# Autodesk Inventor assembly: Grundplatte_test
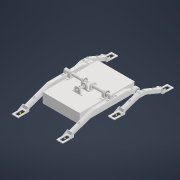
[picture p0: Inventor's stored thumbnail of the model, 180x180]
Saved by Autodesk Inventor 2021 (Build 250183000, 183)
## iProperties
Created: 2021-01-26
Part Number: Grundplatte_test
Document SubType Name: Assembly
Designer: Ctroi
Author: Ctroi
## Documents named in this file (22)
- G:\Roverprojekt\Github Projekt\Rover\Grundplatte_test.iam
- G:\Roverprojekt\Github Projekt\Rover\Grundplatte_hinten.ipt
- G:\Roverprojekt\Github Projekt\Rover\Grundplatte_vorne.ipt
- G:\Roverprojekt\Github Projekt\Rover\ArduinoMega.ipt
- G:\Roverprojekt\Github Projekt\Rover\Relais.ipt
- G:\Roverprojekt\Github Projekt\Rover\Kreuz_Halterung.ipt
- G:\Roverprojekt\Github Projekt\Rover\Obenplatte_hinten.ipt
- G:\Roverprojekt\Github Projekt\Rover\Obenplatte_vorne.ipt
- G:\Roverprojekt\Github Projekt\Rover\Halterung_Differential_3.ipt
- G:\Roverprojekt\Github Projekt\Rover\Halterung_Differential_Mitte.ipt
- G:\Roverprojekt\Github Projekt\Rover\Halterung_Differential.ipt
- G:\Roverprojekt\Github Projekt\Rover\Halterung_Differential_2.ipt
- G:\Roverprojekt\Github Projekt\Rover\Kugellager.ipt
- G:\Roverprojekt\Github Projekt\Rover\Kugellager_klein.ipt
- G:\Roverprojekt\Github Projekt\Rover\Verbindung_Rocker_Body.ipt
- G:\Roverprojekt\Github Projekt\Rover\Welle_Kugellager_Mitte.ipt
- G:\Roverprojekt\Github Projekt\Rover\Rocker_hinten_rechts.ipt
- G:\Roverprojekt\Github Projekt\Rover\Rocker_hinten.ipt
- G:\Roverprojekt\Github Projekt\Rover\Rocker_vorne.ipt
- G:\Roverprojekt\Github Projekt\Rover\Bogie.ipt
- G:\Roverprojekt\Github Projekt\Rover\Boogie_Stange.ipt
- G:\Roverprojekt\Github Projekt\Rover\Servohalterung_v2.ipt
## Components (40 placed, 20 different names)
1. Fahrwerk_bogie:1 — Passend:70, Passend:71, Fluchtend:5, Fluchtend:6, Passend:72, Fluchtend:7, Fluchtend:8, Passend:73
2. Fahrwerk_bogie:2 — Passend:68, Passend:69, Fluchtend:13, Fluchtend:14, Passend:76, Fluchtend:15, Fluchtend:16, Passend:77
3. Boogie_Stange:1 — Passend:64, Passend:65, Passend:68, Passend:69
4. Boogie_Stange:2 — Passend:66, Passend:67, Passend:70, Passend:71
5. Servohalterung_v2:1 — Fluchtend:9, Fluchtend:10, Passend:74
6. Servohalterung_v2:2 — Fluchtend:11, Fluchtend:12, Passend:75
7. Servohalterung_v2:3 — Fluchtend:13, Fluchtend:14, Passend:76
8. Servohalterung_v2:4 — Fluchtend:7, Fluchtend:8, Passend:73
9. Servohalterung_v2:5 — Fluchtend:15, Fluchtend:16, Passend:77
10. Servohalterung_v2:6 — Fluchtend:5, Fluchtend:6, Passend:72
11. Grundplatte_hinten:1 — Passend:1, Passend:2, Passend:5, Passend:6, Passend:7, Passend:11, Passend:12, Passend:13, Passend:16
12. Grundplatte_vorne:1 — Passend:1, Passend:2, Passend:3, Passend:4, Passend:8, Passend:9, Passend:10, Passend:16
13. ArduinoMega:1 — Passend:3, Passend:4
14. Relais:1
15. Kreuz_Halterung:1 — Passend:5, Passend:6, Passend:7
16. Welle_Kugellager_Mitte:1 — Passend:48, Passend:49
17. Obenplatte_vorne:1 — Passend:8, Passend:9, Passend:10, Passend:15, Passend:17, Passend:18, Passend:21, Passend:22, Passend:23, Passend:24, Passend:27, Passend:28
18. Halterung_Differential_3:1 — Passend:14, Passend:15, Passend:17, Passend:38, Passend:39
19. Halterung_Differential_3:2 — Passend:18, Passend:19, Passend:20, Passend:32, Passend:33
20. Obenplatte_hinten:1 — Passend:11, Passend:12, Passend:13, Passend:14, Passend:19, Passend:20, Passend:25, Passend:26
21. Halterung_Differential_Mitte:1 — Passend:21, Passend:22, Passend:23, Passend:42, Passend:43
22. Halterung_Differential:1 — Passend:26, Passend:27, Passend:28, Passend:30, Passend:31, Passend:36, Passend:37
23. Halterung_Differential:2 — Passend:24, Passend:25, Passend:29, Passend:34, Passend:35
24. Halterung_Differential_2:1 — Passend:29, Passend:30, Passend:31, Passend:40, Passend:41
25. Kugellager:1 — Passend:40, Passend:41, Passend:48, Passend:49
26. Kugellager:2 — Passend:32, Passend:33, Passend:47
27. Kugellager:3 — Passend:34, Passend:35, Passend:44
28. Kugellager:4 — Passend:36, Passend:37, Passend:45
29. Kugellager:5 — Passend:38, Passend:39, Passend:46
30. Kugellager_klein:1 — Passend:42, Passend:43
31. Fahrwerk_rocker_vorne:1 — Fluchtend:1, Fluchtend:2, Passend:62, Fluchtend:11, Fluchtend:12, Passend:75
32. Kugellager:7 — Passend:54, Passend:55, Passend:64, Passend:65
33. Kugellager:6 — Passend:52, Passend:53
34. Fahrwerk_rocker_hinten:1 — Passend:50, Passend:51, Passend:52, Passend:53, Passend:54, Passend:55, Fluchtend:1, Fluchtend:2, Passend:62
35. Verbindung_Rocker_Body:1 — Passend:44, Passend:47, Passend:50, Passend:51
36. Kugellager:9 — Passend:60, Passend:61
37. Kugellager:8 — Passend:58, Passend:59, Passend:66, Passend:67
38. Fahrwerk_rocker_hinten:2 — Passend:56, Passend:57, Passend:58, Passend:59, Passend:60, Passend:61, Fluchtend:3, Fluchtend:4, Passend:63
39. Fahrwerk_rocker_vorne:2 — Fluchtend:3, Fluchtend:4, Passend:63, Fluchtend:9, Fluchtend:10, Passend:74
40. Verbindung_Rocker_Body:2 — Passend:45, Passend:46, Passend:56, Passend:57
## Relationships (93: Mate 77, Flush 16)
- Passend:1 [Mate]: Grundplatte_hinten:1 ↔ Grundplatte_vorne:1
- Passend:2 [Mate]: Grundplatte_hinten:1 ↔ Grundplatte_vorne:1
- Passend:3 [Mate]: Grundplatte_vorne:1 ↔ ArduinoMega:1
- Passend:4 [Mate]: Grundplatte_vorne:1 ↔ ArduinoMega:1
- Passend:5 [Mate]: Grundplatte_hinten:1 ↔ Kreuz_Halterung:1
- Passend:6 [Mate]: Grundplatte_hinten:1 ↔ Kreuz_Halterung:1
- Passend:7 [Mate]: Grundplatte_hinten:1 ↔ Kreuz_Halterung:1
- Passend:8 [Mate]: Grundplatte_vorne:1 ↔ Obenplatte_vorne:1
- Passend:9 [Mate]: Grundplatte_vorne:1 ↔ Obenplatte_vorne:1
- Passend:10 [Mate]: Grundplatte_vorne:1 ↔ Obenplatte_vorne:1
- Passend:11 [Mate]: Grundplatte_hinten:1 ↔ Obenplatte_hinten:1
- Passend:12 [Mate]: Grundplatte_hinten:1 ↔ Obenplatte_hinten:1
- Passend:13 [Mate]: Grundplatte_hinten:1 ↔ Obenplatte_hinten:1
- Passend:14 [Mate]: Halterung_Differential_3:1 ↔ Obenplatte_hinten:1
- Passend:15 [Mate]: Obenplatte_vorne:1 ↔ Halterung_Differential_3:1
- Passend:16 [Mate]: Grundplatte_hinten:1 ↔ Grundplatte_vorne:1
- Passend:17 [Mate]: Obenplatte_vorne:1 ↔ Halterung_Differential_3:1
- Passend:18 [Mate]: Obenplatte_vorne:1 ↔ Halterung_Differential_3:2
- Passend:19 [Mate]: Halterung_Differential_3:2 ↔ Obenplatte_hinten:1
- Passend:20 [Mate]: Halterung_Differential_3:2 ↔ Obenplatte_hinten:1
- Passend:21 [Mate]: Obenplatte_vorne:1 ↔ Halterung_Differential_Mitte:1
- Passend:22 [Mate]: Obenplatte_vorne:1 ↔ Halterung_Differential_Mitte:1
- Passend:23 [Mate]: Obenplatte_vorne:1 ↔ Halterung_Differential_Mitte:1
- Passend:24 [Mate]: Obenplatte_vorne:1 ↔ Halterung_Differential:2
- Passend:25 [Mate]: Obenplatte_hinten:1 ↔ Halterung_Differential:2
- Passend:26 [Mate]: Obenplatte_hinten:1 ↔ Halterung_Differential:1
- Passend:27 [Mate]: Obenplatte_vorne:1 ↔ Halterung_Differential:1
- Passend:28 [Mate]: Obenplatte_vorne:1 ↔ Halterung_Differential:1
- Passend:29 [Mate]: Halterung_Differential:2 ↔ Halterung_Differential_2:1
- Passend:30 [Mate]: Halterung_Differential:1 ↔ Halterung_Differential_2:1
- Passend:31 [Mate]: Halterung_Differential:1 ↔ Halterung_Differential_2:1
- Passend:32 [Mate]: Halterung_Differential_3:2 ↔ Kugellager:2
- Passend:33 [Mate]: Halterung_Differential_3:2 ↔ Kugellager:2
- Passend:34 [Mate]: Halterung_Differential:2 ↔ Kugellager:3
- Passend:35 [Mate]: Halterung_Differential:2 ↔ Kugellager:3
- Passend:36 [Mate]: Halterung_Differential:1 ↔ Kugellager:4
- Passend:37 [Mate]: Halterung_Differential:1 ↔ Kugellager:4
- Passend:38 [Mate]: Halterung_Differential_3:1 ↔ Kugellager:5
- Passend:39 [Mate]: Halterung_Differential_3:1 ↔ Kugellager:5
- Passend:40 [Mate]: Halterung_Differential_2:1 ↔ Kugellager:1
- Passend:41 [Mate]: Halterung_Differential_2:1 ↔ Kugellager:1
- Passend:42 [Mate]: Halterung_Differential_Mitte:1 ↔ Kugellager_klein:1
- Passend:43 [Mate]: Halterung_Differential_Mitte:1 ↔ Kugellager_klein:1
- Passend:44 [Mate]: Kugellager:3 ↔ Verbindung_Rocker_Body:1
- Passend:45 [Mate]: Kugellager:4 ↔ Verbindung_Rocker_Body:2
- Passend:46 [Mate]: Kugellager:5 ↔ Verbindung_Rocker_Body:2
- Passend:47 [Mate]: Kugellager:2 ↔ Verbindung_Rocker_Body:1
- Passend:48 [Mate]: Welle_Kugellager_Mitte:1 ↔ Kugellager:1
- Passend:49 [Mate]: Welle_Kugellager_Mitte:1 ↔ Kugellager:1
- Passend:50 [Mate]: Fahrwerk_rocker_hinten:1 ↔ Verbindung_Rocker_Body:1
- Passend:51 [Mate]: Fahrwerk_rocker_hinten:1 ↔ Verbindung_Rocker_Body:1
- Passend:52 [Mate]: Kugellager:6 ↔ Fahrwerk_rocker_hinten:1
- Passend:53 [Mate]: Kugellager:6 ↔ Fahrwerk_rocker_hinten:1
- Passend:54 [Mate]: Kugellager:7 ↔ Fahrwerk_rocker_hinten:1
- Passend:55 [Mate]: Kugellager:7 ↔ Fahrwerk_rocker_hinten:1
- Passend:56 [Mate]: Fahrwerk_rocker_hinten:2 ↔ Verbindung_Rocker_Body:2
- Passend:57 [Mate]: Fahrwerk_rocker_hinten:2 ↔ Verbindung_Rocker_Body:2
- Passend:58 [Mate]: Kugellager:8 ↔ Fahrwerk_rocker_hinten:2
- Passend:59 [Mate]: Kugellager:8 ↔ Fahrwerk_rocker_hinten:2
- Passend:60 [Mate]: Kugellager:9 ↔ Fahrwerk_rocker_hinten:2
- Passend:61 [Mate]: Kugellager:9 ↔ Fahrwerk_rocker_hinten:2
- Fluchtend:1 [Flush]: Fahrwerk_rocker_vorne:1 ↔ Fahrwerk_rocker_hinten:1
- Fluchtend:2 [Flush]: Fahrwerk_rocker_vorne:1 ↔ Fahrwerk_rocker_hinten:1
- Passend:62 [Mate]: Fahrwerk_rocker_vorne:1 ↔ Fahrwerk_rocker_hinten:1
- Fluchtend:3 [Flush]: Fahrwerk_rocker_hinten:2 ↔ Fahrwerk_rocker_vorne:2
- Fluchtend:4 [Flush]: Fahrwerk_rocker_hinten:2 ↔ Fahrwerk_rocker_vorne:2
- Passend:63 [Mate]: Fahrwerk_rocker_hinten:2 ↔ Fahrwerk_rocker_vorne:2
- Passend:64 [Mate]: Boogie_Stange:1 ↔ Kugellager:7
- Passend:65 [Mate]: Boogie_Stange:1 ↔ Kugellager:7
- Passend:66 [Mate]: Boogie_Stange:2 ↔ Kugellager:8
- Passend:67 [Mate]: Boogie_Stange:2 ↔ Kugellager:8
- Passend:68 [Mate]: Fahrwerk_bogie:2 ↔ Boogie_Stange:1
- Passend:69 [Mate]: Fahrwerk_bogie:2 ↔ Boogie_Stange:1
- Passend:70 [Mate]: Fahrwerk_bogie:1 ↔ Boogie_Stange:2
- Passend:71 [Mate]: Fahrwerk_bogie:1 ↔ Boogie_Stange:2
- Fluchtend:5 [Flush]: Fahrwerk_bogie:1 ↔ Servohalterung_v2:6
- Fluchtend:6 [Flush]: Fahrwerk_bogie:1 ↔ Servohalterung_v2:6
- Passend:72 [Mate]: Fahrwerk_bogie:1 ↔ Servohalterung_v2:6
- Fluchtend:7 [Flush]: Fahrwerk_bogie:1 ↔ Servohalterung_v2:4
- Fluchtend:8 [Flush]: Fahrwerk_bogie:1 ↔ Servohalterung_v2:4
- Passend:73 [Mate]: Fahrwerk_bogie:1 ↔ Servohalterung_v2:4
- Fluchtend:9 [Flush]: Servohalterung_v2:1 ↔ Fahrwerk_rocker_vorne:2
- Fluchtend:10 [Flush]: Servohalterung_v2:1 ↔ Fahrwerk_rocker_vorne:2
- Passend:74 [Mate]: Servohalterung_v2:1 ↔ Fahrwerk_rocker_vorne:2
- Fluchtend:11 [Flush]: Servohalterung_v2:2 ↔ Fahrwerk_rocker_vorne:1
- Fluchtend:12 [Flush]: Servohalterung_v2:2 ↔ Fahrwerk_rocker_vorne:1
- Passend:75 [Mate]: Servohalterung_v2:2 ↔ Fahrwerk_rocker_vorne:1
- Fluchtend:13 [Flush]: Fahrwerk_bogie:2 ↔ Servohalterung_v2:3
- Fluchtend:14 [Flush]: Fahrwerk_bogie:2 ↔ Servohalterung_v2:3
- Passend:76 [Mate]: Fahrwerk_bogie:2 ↔ Servohalterung_v2:3
- Fluchtend:15 [Flush]: Fahrwerk_bogie:2 ↔ Servohalterung_v2:5
- Fluchtend:16 [Flush]: Fahrwerk_bogie:2 ↔ Servohalterung_v2:5
- Passend:77 [Mate]: Fahrwerk_bogie:2 ↔ Servohalterung_v2:5
